# Autodesk Inventor assembly: Supershifter Long Hex Wheel Shaft subassembly
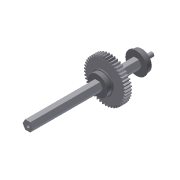
[picture p0: Inventor's stored thumbnail of the model, 180x180]
Saved by Autodesk Inventor 2011 (Build 150239000, 239)
## iProperties
Created: 2012-06-03
Part Number: Supershifter Long Hex Wheel Shaft subassembly
Document SubType Name: Assembly
Designer: Nemo
Author: Nemo
## Documents named in this file (5)
- H:\Nemo\Documents\Robotics\COTS Parts\Gearboxes\Shafts\Supershifter Long Hex Wheel Shaft subassembly.iam
- H:\Nemo\Documents\Robotics\COTS Parts\Gearboxes\Shafts\Supershifter Long Hex Output Shaft.ipt
- H:\Nemo\Documents\Robotics\COTS Parts\Gearboxes\Bearings\Bearing FR8zz.ipt
- H:\Nemo\Documents\Robotics\COTS Parts\Gearboxes\Gears\Gear 20dp 500hex 45T.ipt
- H:\Nemo\Documents\Robotics\COTS Parts\Gearboxes\Bearings\Bearing FR8zz-hex.ipt
## Components (4 placed, 4 different names)
1. Supershifter Long Hex Output Shaft:1 — Insert:1, Mate:1, Angle:1, Mate:2, Angle:2
2. Bearing FR8zz:1 — Insert:1, Mate:3
3. Gear 45T 20dp 500hex:1 — Mate:1, Angle:1
4. Bearing FR8zz-hex:1 — Mate:2, Angle:2, Mate:3
## Relationships (6: Mate 3, Angle 2, Insert 1)
- Insert:1: Supershifter Long Hex Output Shaft:1 ↔ Bearing FR8zz:1
- Mate:1: Supershifter Long Hex Output Shaft:1 ↔ Gear 45T 20dp 500hex:1
- Angle:1 (0 deg): Supershifter Long Hex Output Shaft:1 ↔ Gear 45T 20dp 500hex:1
- Mate:2: Supershifter Long Hex Output Shaft:1 ↔ Bearing FR8zz-hex:1
- Angle:2 (0 deg): Supershifter Long Hex Output Shaft:1 ↔ Bearing FR8zz-hex:1
- Mate:3 (-50.8 mm): Bearing FR8zz:1 ↔ Bearing FR8zz-hex:1
